# Autodesk Inventor assembly: 0_Entire_Assembly
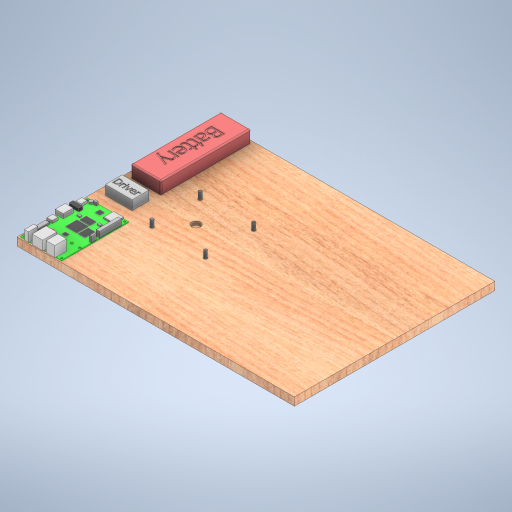
[picture p0: Inventor's stored thumbnail of the model, 512x512]
Saved by Autodesk Inventor 2024.2 (Build 282272000, 272)
## iProperties
Created: 2023-08-24
Part Number: 0_Entire_Assembly
Document SubType Name: Assembly
Designer: chanh
Author: chanh
## Documents named in this file (6)
- C:\Users\chanh\내 드라이브\로봇\Humanoid\Roboin Humanoid Project\Inventor\rh_plus_7_axis_robot_arm_hardware\Assembly\1_Base.iam
- C:\Users\chanh\내 드라이브\로봇\Humanoid\Roboin Humanoid Project\Inventor\rh_plus_7_axis_robot_arm_hardware\Part\Other Parts\base_plate.ipt
- C:\Users\chanh\내 드라이브\로봇\Humanoid\Roboin Humanoid Project\Inventor\rh_plus_7_axis_robot_arm_hardware\Part\Bolt, Bearing, Nut, Washer\M5x22 Flat Head Bolt.ipt
- C:\Users\chanh\내 드라이브\로봇\Humanoid\Roboin Humanoid Project\Inventor\rh_plus_7_axis_robot_arm_hardware\Part\Other Parts\orange pi5.iam
- C:\Users\chanh\내 드라이브\로봇\Humanoid\Roboin Humanoid Project\Inventor\rh_plus_7_axis_robot_arm_hardware\Part\Other Parts\Battery_Pack.ipt
- C:\Users\chanh\내 드라이브\로봇\Humanoid\Roboin Humanoid Project\Inventor\rh_plus_7_axis_robot_arm_hardware\Part\Other Parts\Motor_Driver.ipt
## Components (8 placed, 5 different names)
1. base_plate:1 — Flush:1, Flush:2, Flush:3, Rigid:1, Rigid:2, Rigid:3, Rigid:4, Mate:1, Flush:4, Flush:5, Mate:2, Flush:6, Flush:7, Mate:3, Flush:8
2. M5x22 Flat Head Bolt:1 — Rigid:3
3. M5x22 Flat Head Bolt:2 — Rigid:4
4. M5x22 Flat Head Bolt:3 — Rigid:1
5. M5x22 Flat Head Bolt:4 — Rigid:2
6. orange pi5:1 [sub-assembly] — Mate:1, Flush:4, Flush:5
7. Battery_Pack:1 — Mate:2, Flush:6, Flush:7, Mate:4
8. Motor_Driver:1 — Mate:3, Flush:8, Mate:4
## Relationships (16: Flush 8, WeldJoint 4, Mate 4)
- Flush:1: base_plate:1
- Flush:2: base_plate:1
- Flush:3: base_plate:1
- Rigid:1 [WeldJoint]: base_plate:1 ↔ M5x22 Flat Head Bolt:3
- Rigid:2 [WeldJoint]: base_plate:1 ↔ M5x22 Flat Head Bolt:4
- Rigid:3 [WeldJoint]: base_plate:1 ↔ M5x22 Flat Head Bolt:1
- Rigid:4 [WeldJoint]: base_plate:1 ↔ M5x22 Flat Head Bolt:2
- Mate:1: base_plate:1 ↔ orange pi5:1
- Flush:4: base_plate:1 ↔ orange pi5:1
- Flush:5: base_plate:1 ↔ orange pi5:1
- Mate:2: base_plate:1 ↔ Battery_Pack:1
- Flush:6 (10 mm): base_plate:1 ↔ Battery_Pack:1
- Flush:7 (5 mm): base_plate:1 ↔ Battery_Pack:1
- Mate:3: base_plate:1 ↔ Motor_Driver:1
- Flush:8 (12 mm): base_plate:1 ↔ Motor_Driver:1
- Mate:4 (15 mm): Battery_Pack:1 ↔ Motor_Driver:1
